# Autodesk Inventor assembly: 000 Ensamblaje hw_LM - BASIC
(part 3 of 3)
- Angle:141 (0 deg): S32E288ABCAAMJGT:1 ↔ UQFN-16:2
## Named parameters: d177_d162 = 0 mm, d178_d163 = 0 mm, d182_d178_d163 = 0 mm, d183_d180 = 0 mm, d191_d186 = 0 mm, d192_d187 = 0 mm, d193_d188 = 0 mm, d194_d189 = 0 mm, d196_d184 = 0 mm, d197_d177_d162 = 0 mm, d198_d178_d163 = 0 mm, d199_d179 = 0 mm, d200_d180 = 0 mm, d201_d184 = 0 mm, d202_d177_d162 = 0 mm, d203_d178_d163 = 0 mm, d204_d179 = 0 mm, d205_d180 = 0 mm, d230_d186 = 0 mm, d231_d187 = 0 mm, d237_d198_d178_d163 = 0 mm, d238_d200_d180 = 0 mm, d239_d202_d177_d162 = 0 mm, d240_d203_d178_d163 = 0 mm, d241_d204_d179 = 0 mm, d242_d205_d180 = 0 mm, d243_d206 = 0 mm, d264_d261 = 0 mm, d265_d262 = 0 mm, d266_d263 = 0 mm, d304_d302 = 0 mm, d308_d306 = 0 mm, d309_d307 = 0 mm, d310_d304_d302 = 0 mm, d312_d306 = 0 mm, d313_d307 = 0 mm, d314_d304_d302 = 0 mm, d316_d237_d198_d178_d163 = 0 mm, d317_d238_d200_d180 = 0 mm, d318_d240_d203_d178_d163 = 0 mm, d319_d242_d205_d180 = 0 mm, d320_d243_d206 = 0 mm, d323_d316_d237_d198_d178_d163 = 0 mm, d324_d317_d238_d200_d180 = 0 mm, d325_d318_d240_d203_d178_d163 = 0 mm, d326_d319_d242_d205_d180 = 0 mm, d327_d320_d243_d206 = 0 mm, d328_d321 = 0 mm, d331_d323_d316_d237_d198_d178_d163 = 0 mm, d332_d324_d317_d238_d200_d180 = 0 mm, d336_d306 = 0 mm, d337_d322 = 0 mm, d338_d304_d302 = 0 mm, d345_d237_d198_d178_d163 = 0 mm, d346_d238_d200_d180 = 0 mm, d398_d394 = 0 mm, d399_d395 = 0 mm, d421_d415 = 0 mm, d442_d178_d163 = 0 mm, d443_d180 = 0 mm, d444_d178_d163 = 0 mm, d445_d180 = 0 mm, d446_d178_d163 = 0 mm, d447_d180 = 0 mm, d456_d340 = 0 mm, d457_d340 = 0 mm, d463_d456_d340 = 0 mm, d464_d457_d340 = 0 mm, d465_d458 = 0 mm, d466_d459 = 0 mm, d467_d460 = 0 mm, d468_d461 = 0 mm, d471_d456_d340 = 0 mm, d472_d457_d340 = 0 mm, d473_d458 = 0 mm, d474_d459 = 0 mm, d475_d460 = 0 mm, d476_d461 = 0 mm, d477_d463_d456_d340 = 0 mm, d478_d464_d457_d340 = 0 mm, d479_d465_d458 = 0 mm, d480_d466_d459 = 0 mm, d481_d467_d460 = 0 mm, d482_d468_d461 = 0 mm, d483_d469 = 0 mm, d484_d470 = 0 mm, d488_d471_d456_d340 = 0 mm, d489_d472_d457_d340 = 0 mm, d490_d473_d458 = 0 mm, d491_d474_d459 = 0 mm, d492_d475_d460 = 0 mm, d493_d476_d461 = 0 mm, d494_d477_d463_d456_d340 = 0 mm, d495_d478_d464_d457_d340 = 0 mm, d496_d479_d465_d458 = 0 mm, d497_d480_d466_d459 = 0 mm, d498_d481_d467_d460 = 0 mm, d499_d482_d468_d461 = 0 mm, d500_d483_d469 = 0 mm, d501_d484_d470 = 0 mm, d502_d486 = 0 mm, d506_d471_d456_d340 = 0 mm, d507_d489_d472_d457_d340 = 0 mm, d508_d490_d473_d458 = 0 mm, d509_d492_d475_d460 = 0 mm, d510_d495_d478_d464_d457_d340 = 0 mm, d511_d496_d479_d465_d458 = 0 mm, d512_d498_d481_d467_d460 = 0 mm, d513_d502_d486 = 0 mm, d514_d503 = 0 mm, d515_d504 = 0 mm, d516_d471_d456_d340 = 0 mm, d517_d489_d472_d457_d340 = 0 mm, d518_d490_d473_d458 = 0 mm, d519_d492_d475_d460 = 0 mm, d520_d495_d478_d464_d457_d340 = 0 mm, d521_d496_d479_d465_d458 = 0 mm, d522_d498_d481_d467_d460 = 0 mm, d523_d502_d486 = 0 mm, d524_d503 = 0 mm, d525_d504 = 0 mm, d529_d507_d489_d472_d457_d340 = 0 mm, d530_d508_d490_d473_d458 = 0 mm, d531_d509_d492_d475_d460 = 0 mm, d575_d507_d489_d472_d457_d340 = 0 mm, d576_d508_d490_d473_d458 = 0 mm, d577_d509_d492_d475_d460 = 0 mm, d581_d575_d507_d489_d472_d457_d340 = 0 mm, d582_d576_d508_d490_d473_d458 = 0 mm, d583_d577_d509_d492_d475_d460 = 0 mm, d584_d578 = 0 mm, d585_d579 = 0 mm, d586_d580 = 0 mm, d591_d581_d575_d507_d489_d472_d457_d340 = 0 mm, d592_d582_d576_d508_d490_d473_d458 = 0 mm, d593_d583_d577_d509_d492_d475_d460 = 0 mm, d594_d584_d578 = 0 mm, d595_d585_d579 = 0 mm, d596_d586_d580 = 0 mm, d597_d589 = 0 mm, d598_d590 = 0 mm, d599_d581_d575_d507_d489_d472_d457_d340 = 0 mm, d600_d582_d576_d508_d490_d473_d458 = 0 mm, d601_d583_d577_d509_d492_d475_d460 = 0 mm, d602_d584_d578 = 0 mm, d603_d585_d579 = 0 mm, d604_d586_d580 = 0 mm, d605_d589 = 0 mm, d606_d590 = 0 mm, d607_d591_d581_d575_d507_d489_d472_d457_d340 = 0 mm, d608_d592_d582_d576_d508_d490_d473_d458 = 0 mm, d609_d593_d583_d577_d509_d492_d475_d460 = 0 mm, d610_d594_d584_d578 = 0 mm, d611_d595_d585_d579 = 0 mm, d612_d596_d586_d580 = 0 mm, d613_d597_d589 = 0 mm, d614_d598_d590 = 0 mm, d632_d599_d581_d575_d507_d489_d472_d457_d340 = 0 mm, d633_d600_d582_d576_d508_d490_d473_d458 = 0 mm, d634_d601_d583_d577_d509_d492_d475_d460 = 0 mm, d635_d602_d584_d578 = 0 mm, d636_d603_d585_d579 = 0 mm, d637_d604_d586_d580 = 0 mm, d638_d605_d589 = 0 mm, d639_d606_d590 = 0 mm, d640_d623 = 0 deg, d641_d624 = 0 deg, d642_d625 = 0 deg, d643_d626 = 0 deg, d644_d627 = 0 deg, d645_d628 = 0 deg, d646_d629 = 0 deg, d650_d581_d575_d507_d489_d472_d457_d340 = 0 mm, d651_d582_d576_d508_d490_d473_d458 = 0 mm, d652_d446_d178_d163 = 0 mm, d653_d447_d180 = 0 mm, d654_d449 = 0 mm, d655_d452 = 0 mm, d656_d581_d575_d507_d489_d472_d457_d340 = 0 mm, d657_d582_d576_d508_d490_d473_d458 = 0 mm, d658_d446_d178_d163 = 0 mm, d659_d447_d180 = 0 mm, d660_d449 = 0 mm, d661_d452 = 0 mm, d671_d574 = 0 mm, d682_d678 = 0 mm, d683_d679 = 0 mm, d684_d680 = 0 mm, d709_d706 = 0 mm, d710_d707 = 0 mm, d733_d728 = 0 mm, d734_d730 = 0 mm, d735_d731 = 0 mm, d736_d732 = 0 mm, d737_d728 = 0 mm, d738_d730 = 0 mm, d739_d731 = 0 mm, d740_d732 = 0 mm, d746_d737_d728 = 0 mm, d747_d738_d730 = 0 mm, d748_d739_d731 = 0 mm, d749_d740_d732 = 0 mm, d750_d737_d728 = 0 mm, d751_d738_d730 = 0 mm, d752_d739_d731 = 0 mm, d753_d740_d732 = 0 mm, d759_d750_d737_d728 = 0 mm, d760_d751_d738_d730 = 0 mm, d761_d752_d739_d731 = 0 mm, d762_d753_d740_d732 = 0 mm, d763_d750_d737_d728 = 0 mm, d764_d751_d738_d730 = 0 mm, d765_d752_d739_d731 = 0 mm, d766_d753_d740_d732 = 0 mm, d771_d763_d750_d737_d728 = 0 mm, d772_d764_d751_d738_d730 = 0 mm, d773_d765_d752_d739_d731 = 0 mm, d774_d766_d753_d740_d732 = 0 mm, d775_d763_d750_d737_d728 = 0 mm, d776_d764_d751_d738_d730 = 0 mm, d777_d765_d752_d739_d731 = 0 mm, d778_d766_d753_d740_d732 = 0 mm, d783_d775_d763_d750_d737_d728 = 0 mm, d784_d777_d765_d752_d739_d731 = 0 mm, d785_d778_d766_d753_d740_d732 = 0 mm, d786_d775_d763_d750_d737_d728 = 0 mm, d787_d777_d765_d752_d739_d731 = 0 mm, d788_d778_d766_d753_d740_d732 = 0 mm, d798_d775_d763_d750_d737_d728 = 0 mm, d799_d786_d775_d763_d750_d737_d728 = 0 mm, d800_d787_d777_d765_d752_d739_d731 = 0 mm, d801_d788_d778_d766_d753_d740_d732 = 0 mm, d802_d790 = 0 deg, d803_d793 = 0 deg, d804_d794 = 0 deg, d810_d786_d775_d763_d750_d737_d728 = 0 mm, d811_d787_d777_d765_d752_d739_d731 = 0 mm, d812_d788_d778_d766_d753_d740_d732 = 0 mm, d814_d793 = 0 deg, d815_d794 = 0 deg, d816_d798_d775_d763_d750_d737_d728 = 0 mm, d817_d799_d786_d775_d763_d750_d737_d728 = 0 mm, d818_d800_d787_d777_d765_d752_d739_d731 = 0 mm, d819_d801_d788_d778_d766_d753_d740_d732 = 0 mm, d820_d802_d790 = 0 deg, d821_d803_d793 = 0 deg, d822_d804_d794 = 0 deg, d823_d805 = 0 mm, d824_d806 = 0 mm, d825_d807 = 0 mm, d836_d829 = 0 mm, d839_d810_d786_d775_d763_d750_d737_d728 = 0 mm, d840_d811_d787_d777_d765_d752_d739_d731 = 0 mm, d841_d812_d788_d778_d766_d753_d740_d732 = 0 mm, d842_d814_d793 = 0 deg, d843_d815_d794 = 0 deg, d844_d817_d799_d786_d775_d763_d750_d737_d728 = 0 mm, d845_d818_d800_d787_d777_d765_d752_d739_d731 = 0 mm, d846_d819_d801_d788_d778_d766_d753_d740_d732 = 0 mm, d847_d821_d803_d793 = 0 deg, d848_d822_d804_d794 = 0 deg, d856_d836_d829 = 0 mm, d857_d837_d775_d763_d750_d737_d728 = 0 mm, d858_d838_d790 = 0 deg, d859_d839_d810_d786_d775_d763_d750_d737_d728 = 0 mm, d860_d840_d811_d787_d777_d765_d752_d739_d731 = 0 mm, d861_d841_d812_d788_d778_d766_d753_d740_d732 = 0 mm, d862_d842_d814_d793 = 0 deg, d863_d843_d815_d794 = 0 deg, d867_d847_d821_d803_d793 = 0 deg, d868_d848_d822_d804_d794 = 0 deg, d869_d849 = 0 mm, d870_d851 = 0 mm, d871_d852 = 0 mm, d872_d853 = 0 mm, d880_d878 = 0 deg, d882_d847_d821_d803_d793 = 0 deg, d886_d883 = 0 mm, d887_d884 = 0 mm, d888_d885 = 0 mm, d889_d878 = 0 deg, d890_d880_d878 = 0 deg, d892_d882_d847_d821_d803_d793 = 0 deg, d894_d847_d821_d803_d793 = 0 deg, d899_d878 = 0 deg, d901_d847_d821_d803_d793 = 0 deg, d906_d878 = 0 deg, d908_d847_d821_d803_d793 = 0 deg
